# Autodesk Inventor assembly: MotorMountAssembly
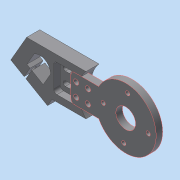
[picture p0: Inventor's stored thumbnail of the model, 180x180]
Saved by Autodesk Inventor 2017 (Build 210142000, 142)
## iProperties
Created: 2015-12-28
Part Number: MotorMountAssembly
Document SubType Name: Assembly
Designer: JoshuaYuan
Author: JoshuaYuan
## Documents named in this file (3)
- C:\Other Project Stuff\Longboard\MotorMountAssembly.iam
- C:\Other Project Stuff\Longboard\motormount3.ipt
- C:\Other Project Stuff\Longboard\motormount3_C.ipt
## Components (2 placed, 2 different names)
1. motormount3:1 — Mate:1, Mate:2
2. motormount3_C:1 — Mate:1, Mate:2
## Relationships (2: Mate 2)
- Mate:1: motormount3:1 ↔ motormount3_C:1
- Mate:2: motormount3:1 ↔ motormount3_C:1
